# Autodesk Inventor assembly: Zusammenbau_V3
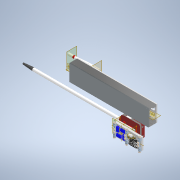
[picture p0: Inventor's stored thumbnail of the model, 180x180]
Saved by Autodesk Inventor 2022 (Build 260153000, 153)
## iProperties
Created: 2022-05-05
Part Number: Zusammenbau_V3
Document SubType Name: Assembly
Designer: 123St
Author: 123St
## Documents named in this file (18)
- C:\Users\alexw\Documents\Inventor\Projects\03_CurrentProjects\MasterThesis\PSM_V1_Rillenkugellager\Ueberarbeiteter DaVincikopf\Zusammenbau_V3.iam
- C:\Users\alexw\Documents\Inventor\Projects\03_CurrentProjects\MasterThesis\PSM_V1_Rillenkugellager\Ueberarbeiteter DaVincikopf\Fuehrungsgrundplatte_V3.ipt
- C:\Users\alexw\Documents\Inventor\Projects\03_CurrentProjects\MasterThesis\PSM_V1_Rillenkugellager\Ueberarbeiteter DaVincikopf\JX BLS-HV7146MG.iam
- C:\Users\alexw\Documents\Inventor\Projects\03_CurrentProjects\MasterThesis\PSM_V1_Rillenkugellager\Ueberarbeiteter DaVincikopf\SG90 - Micro Servo 9g - Tower Pro.iam
- C:\Users\alexw\Documents\Inventor\Projects\03_CurrentProjects\MasterThesis\PSM_V1_Rillenkugellager\Ueberarbeiteter DaVincikopf\Fuehrungslagerhalter_v2.ipt
- C:\Users\alexw\Documents\Inventor\Projects\03_CurrentProjects\MasterThesis\PSM_V1_Rillenkugellager\Ueberarbeiteter DaVincikopf\Adaptation_on_OPdevside_4_2.ipt
- C:\Users\alexw\Documents\Inventor\Projects\03_CurrentProjects\MasterThesis\PSM_V1_Rillenkugellager\Ueberarbeiteter DaVincikopf\Fuehrungsschiene.ipt
- C:\Users\alexw\Documents\Inventor\Projects\03_CurrentProjects\MasterThesis\PSM_V1_Rillenkugellager\Ueberarbeiteter DaVincikopf\Lager.iam
- C:\Users\alexw\Documents\Inventor\Projects\03_CurrentProjects\MasterThesis\PSM_V1_Rillenkugellager\Ueberarbeiteter DaVincikopf\Zahnradbahn.ipt
- C:\Users\alexw\Documents\Inventor\Projects\03_CurrentProjects\MasterThesis\PSM_V1_Rillenkugellager\Ueberarbeiteter DaVincikopf\Zahnrad.ipt
- C:\Users\alexw\Documents\Inventor\Projects\03_CurrentProjects\MasterThesis\PSM_V1_Rillenkugellager\Ueberarbeiteter DaVincikopf\Op_dev_gehäuse.ipt
- C:\Users\alexw\Documents\Inventor\Projects\03_CurrentProjects\MasterThesis\PSM_V1_Rillenkugellager\Ueberarbeiteter DaVincikopf\Op_dev_stange.ipt
- C:\Users\alexw\Documents\Inventor\Projects\03_CurrentProjects\MasterThesis\PSM_V1_Rillenkugellager\Ueberarbeiteter DaVincikopf\Oberteil_servoplatte.ipt
- C:\Users\alexw\Documents\Inventor\Projects\03_CurrentProjects\MasterThesis\PSM_V1_Rillenkugellager\Ueberarbeiteter DaVincikopf\Adaptation_2.ipt
- C:\Users\alexw\Documents\Inventor\Projects\03_CurrentProjects\MasterThesis\PSM_V1_Rillenkugellager\Ueberarbeiteter DaVincikopf\Adaptation_2_1.ipt
- C:\Users\alexw\Documents\Inventor\Projects\03_CurrentProjects\MasterThesis\PSM_V1_Rillenkugellager\Back plate profile.ipt
- C:\Users\alexw\Documents\Inventor\Projects\03_CurrentProjects\MasterThesis\PSM_V1_Rillenkugellager\Slot profile.ipt
- C:\Users\alexw\Documents\Inventor\Projects\03_CurrentProjects\MasterThesis\PSM_V1_Rillenkugellager\Guide.ipt
## Components (36 placed, 17 different names)
1. Fuehrungsschiene:1 — Passend:21, Passend:37, Passend:38, Passend:39, Passend:40, Passend:46, Passend:47, Passend:48
2. Fuehrungsgrundplatte_V3:1 — Fluchtend:1, Passend:1, Passend:2, Passend:3, Passend:4, Passend:5, Passend:6, Passend:7, Passend:8, Passend:9, Passend:10, Passend:11, Passend:12, Passend:13, Passend:14, Passend:15, Passend:16, Fluchtend:2, Passend:17, Fluchtend:3, Passend:18, Passend:19, Fluchtend:4, Passend:20, Fluchtend:7, Passend:34, Fluchtend:9, Einfügen:1
3. JX BLS-HV7146MG:1 [sub-assembly] — Fluchtend:1, Passend:1, Passend:2, Drehbar:17
4. SG90 - Micro Servo 9g - Tower Pro:2 [sub-assembly] — Passend:6, Passend:11, Passend:12, Drehbar:21
5. SG90 - Micro Servo 9g - Tower Pro:3 [sub-assembly] — Passend:4, Passend:9, Passend:10, Drehbar:22
6. SG90 - Micro Servo 9g - Tower Pro:4 [sub-assembly] — Passend:5, Passend:7, Passend:8, Drehbar:19
7. SG90 - Micro Servo 9g - Tower Pro:5 [sub-assembly] — Passend:3, Passend:13, Passend:14, Fluchtend:6, Drehbar:20
8. Fuehrungslagerhalter_v2:1 — Passend:15, Passend:16, Fluchtend:2, Drehbar:5, Drehbar:10, Drehbar:15, Drehbar:16, Passend:21
9. Fuehrungslagerhalter_v2:2 — Passend:17, Fluchtend:3, Passend:18, Drehbar:6, Drehbar:9, Drehbar:13, Drehbar:14
10. Fuehrungslagerhalter_v2:3 — Passend:19, Fluchtend:4, Passend:20, Drehbar:7, Drehbar:8, Drehbar:11, Drehbar:12
11. Adaptation_on_OPdevside_4_2:1 — Drehbar:21
12. Adaptation_on_OPdevside_4_2:2 — Drehbar:22
13. Adaptation_on_OPdevside_4_2:3 — Drehbar:20
14. Adaptation_on_OPdevside_4_2:4 — Passend:31, Drehbar:19
15. Lager:1 [sub-assembly] — Drehbar:15
16. Lager:2 [sub-assembly] — Drehbar:16
17. Lager:3 [sub-assembly] — Drehbar:13
18. Lager:4 [sub-assembly] — Drehbar:14
19. Lager:5 [sub-assembly] — Drehbar:11
20. Lager:6 [sub-assembly] — Drehbar:12
21. Lager:7 [sub-assembly] — Drehbar:10
22. Lager:8 [sub-assembly] — Drehbar:9
23. Lager:9 [sub-assembly] — Drehbar:8
24. Lager:10 [sub-assembly] — Drehbar:5
25. Lager:11 [sub-assembly] — Drehbar:6
26. Lager:12 [sub-assembly] — Drehbar:7
27. Zahnrad:1 — Drehbar:17
28. Op_dev_gehäuse:1 — Passend:31, Fluchtend:6, Fluchtend:7, Drehbar:18
29. Op_dev_stange:1 — Drehbar:18
30. Oberteil_servoplatte:1 — Passend:34, Fluchtend:9, Einfügen:1, Einfügen:6, Passend:35, Einfügen:7, Passend:36
31. Adaptation_2:1 — Einfügen:6, Passend:35
32. Adaptation_2_1:1 — Einfügen:7, Passend:36
33. Back plate profile:1 — Passend:37, Passend:38
34. Slot profile:1 — Passend:39, Passend:40, Passend:41, Passend:42, Passend:43
35. Guide:1 — Passend:41, Passend:42, Passend:43
36. Zahnradbahn:1 — Passend:46, Passend:47, Passend:48
## Relationships (63: Mate 35, RevoluteJoint 18, Flush 7, Insert 3)
- Fluchtend:1 [Flush] (-5 mm): Fuehrungsgrundplatte_V3:1 ↔ JX BLS-HV7146MG:1
- Passend:1 [Mate]: Fuehrungsgrundplatte_V3:1 ↔ JX BLS-HV7146MG:1
- Passend:2 [Mate]: Fuehrungsgrundplatte_V3:1 ↔ JX BLS-HV7146MG:1
- Passend:3 [Mate]: Fuehrungsgrundplatte_V3:1 ↔ SG90 - Micro Servo 9g - Tower Pro:5
- Passend:4 [Mate]: Fuehrungsgrundplatte_V3:1 ↔ SG90 - Micro Servo 9g - Tower Pro:3
- Passend:5 [Mate]: Fuehrungsgrundplatte_V3:1 ↔ SG90 - Micro Servo 9g - Tower Pro:4
- Passend:6 [Mate]: Fuehrungsgrundplatte_V3:1 ↔ SG90 - Micro Servo 9g - Tower Pro:2
- Passend:7 [Mate] (0.5 mm): Fuehrungsgrundplatte_V3:1 ↔ SG90 - Micro Servo 9g - Tower Pro:4
- Passend:8 [Mate] (0.5 mm): Fuehrungsgrundplatte_V3:1 ↔ SG90 - Micro Servo 9g - Tower Pro:4
- Passend:9 [Mate] (0.5 mm): Fuehrungsgrundplatte_V3:1 ↔ SG90 - Micro Servo 9g - Tower Pro:3
- Passend:10 [Mate] (0.5 mm): Fuehrungsgrundplatte_V3:1 ↔ SG90 - Micro Servo 9g - Tower Pro:3
- Passend:11 [Mate] (0.5 mm): Fuehrungsgrundplatte_V3:1 ↔ SG90 - Micro Servo 9g - Tower Pro:2
- Passend:12 [Mate] (0.5 mm): Fuehrungsgrundplatte_V3:1 ↔ SG90 - Micro Servo 9g - Tower Pro:2
- Passend:13 [Mate] (0.5 mm): Fuehrungsgrundplatte_V3:1 ↔ SG90 - Micro Servo 9g - Tower Pro:5
- Passend:14 [Mate] (0.5 mm): Fuehrungsgrundplatte_V3:1 ↔ SG90 - Micro Servo 9g - Tower Pro:5
- Passend:15 [Mate]: Fuehrungsgrundplatte_V3:1 ↔ Fuehrungslagerhalter_v2:1
- Passend:16 [Mate]: Fuehrungsgrundplatte_V3:1 ↔ Fuehrungslagerhalter_v2:1
- Fluchtend:2 [Flush]: Fuehrungsgrundplatte_V3:1 ↔ Fuehrungslagerhalter_v2:1
- Passend:17 [Mate]: Fuehrungsgrundplatte_V3:1 ↔ Fuehrungslagerhalter_v2:2
- Fluchtend:3 [Flush]: Fuehrungsgrundplatte_V3:1 ↔ Fuehrungslagerhalter_v2:2
- Passend:18 [Mate]: Fuehrungsgrundplatte_V3:1 ↔ Fuehrungslagerhalter_v2:2
- Passend:19 [Mate]: Fuehrungsgrundplatte_V3:1 ↔ Fuehrungslagerhalter_v2:3
- Fluchtend:4 [Flush]: Fuehrungsgrundplatte_V3:1 ↔ Fuehrungslagerhalter_v2:3
- Passend:20 [Mate]: Fuehrungsgrundplatte_V3:1 ↔ Fuehrungslagerhalter_v2:3
- Drehbar:5 [RevoluteJoint]: Fuehrungslagerhalter_v2:1 ↔ Lager:10
- Drehbar:6 [RevoluteJoint]: Fuehrungslagerhalter_v2:2 ↔ Lager:11
- Drehbar:7 [RevoluteJoint]: Fuehrungslagerhalter_v2:3 ↔ Lager:12
- Drehbar:8 [RevoluteJoint]: Fuehrungslagerhalter_v2:3 ↔ Lager:9
- Drehbar:9 [RevoluteJoint]: Fuehrungslagerhalter_v2:2 ↔ Lager:8
- Drehbar:10 [RevoluteJoint]: Fuehrungslagerhalter_v2:1 ↔ Lager:7
- Drehbar:11 [RevoluteJoint]: Fuehrungslagerhalter_v2:3 ↔ Lager:5
- Drehbar:12 [RevoluteJoint]: Fuehrungslagerhalter_v2:3 ↔ Lager:6
- Drehbar:13 [RevoluteJoint]: Fuehrungslagerhalter_v2:2 ↔ Lager:3
- Drehbar:14 [RevoluteJoint]: Fuehrungslagerhalter_v2:2 ↔ Lager:4
- Drehbar:15 [RevoluteJoint]: Fuehrungslagerhalter_v2:1 ↔ Lager:1
- Drehbar:16 [RevoluteJoint]: Fuehrungslagerhalter_v2:1 ↔ Lager:2
- Passend:21 [Mate] (2 mm): Fuehrungsschiene:1 ↔ Fuehrungslagerhalter_v2:1
- Drehbar:17 [RevoluteJoint]: JX BLS-HV7146MG:1 ↔ Zahnrad:1
- Passend:31 [Mate] (15 mm): Adaptation_on_OPdevside_4_2:4 ↔ Op_dev_gehäuse:1
- Fluchtend:6 [Flush] (-25 mm): SG90 - Micro Servo 9g - Tower Pro:5 ↔ Op_dev_gehäuse:1
- Fluchtend:7 [Flush] (-7 mm): Fuehrungsgrundplatte_V3:1 ↔ Op_dev_gehäuse:1
- Drehbar:18 [RevoluteJoint]: Op_dev_gehäuse:1 ↔ Op_dev_stange:1
- Drehbar:19 [RevoluteJoint]: SG90 - Micro Servo 9g - Tower Pro:4 ↔ Adaptation_on_OPdevside_4_2:4
- Drehbar:20 [RevoluteJoint]: SG90 - Micro Servo 9g - Tower Pro:5 ↔ Adaptation_on_OPdevside_4_2:3
- Drehbar:21 [RevoluteJoint]: SG90 - Micro Servo 9g - Tower Pro:2 ↔ Adaptation_on_OPdevside_4_2:1
- Drehbar:22 [RevoluteJoint]: SG90 - Micro Servo 9g - Tower Pro:3 ↔ Adaptation_on_OPdevside_4_2:2
- Passend:34 [Mate]: Fuehrungsgrundplatte_V3:1 ↔ Oberteil_servoplatte:1
- Fluchtend:9 [Flush]: Fuehrungsgrundplatte_V3:1 ↔ Oberteil_servoplatte:1
- Einfügen:1 [Insert]: Fuehrungsgrundplatte_V3:1 ↔ Oberteil_servoplatte:1
- Einfügen:6 [Insert] (-5 mm): Oberteil_servoplatte:1 ↔ Adaptation_2:1
- Passend:35 [Mate]: Oberteil_servoplatte:1 ↔ Adaptation_2:1
- Einfügen:7 [Insert] (-5 mm): Oberteil_servoplatte:1 ↔ Adaptation_2_1:1
- Passend:36 [Mate]: Oberteil_servoplatte:1 ↔ Adaptation_2_1:1
- Passend:37 [Mate]: Fuehrungsschiene:1 ↔ Back plate profile:1
- Passend:38 [Mate]: Fuehrungsschiene:1 ↔ Back plate profile:1
- Passend:39 [Mate]: Fuehrungsschiene:1 ↔ Slot profile:1
- Passend:40 [Mate]: Fuehrungsschiene:1 ↔ Slot profile:1
- Passend:41 [Mate]: Slot profile:1 ↔ Guide:1
- Passend:42 [Mate]: Slot profile:1 ↔ Guide:1
- Passend:43 [Mate]: Slot profile:1 ↔ Guide:1
- Passend:46 [Mate] (11.5 mm): Fuehrungsschiene:1 ↔ Zahnradbahn:1
- Passend:47 [Mate]: Fuehrungsschiene:1 ↔ Zahnradbahn:1
- Passend:48 [Mate]: Fuehrungsschiene:1 ↔ Zahnradbahn:1
